# Autodesk Inventor assembly: Wobbler Assembly
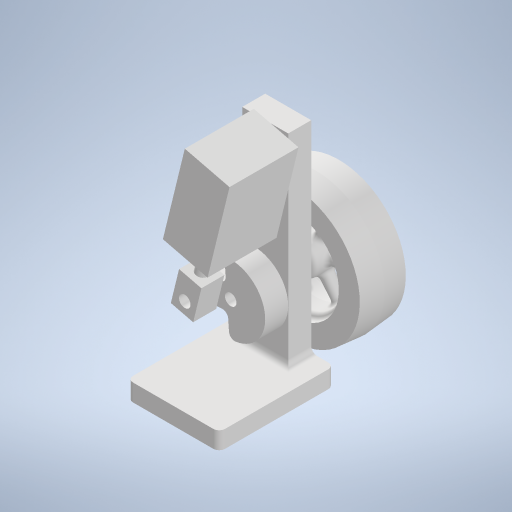
[picture p0: Inventor's stored thumbnail of the model, 512x512]
Saved by Autodesk Inventor 2023 (Build 270158000, 158)
## iProperties
Created: 2022-12-28
Part Number: Wobbler Assembly
Document SubType Name: Assembly
Designer: tgr41
Author: tgr41
## Documents named in this file (6)
- C:\Users\tommy\Documents\Repositories\Steam-Engine\Cast Wobbler\Wobbler Assembly.iam
- C:\Users\tommy\Documents\Repositories\Steam-Engine\Cast Wobbler\Crank.ipt
- C:\Users\tommy\Documents\Repositories\Steam-Engine\Cast Wobbler\Cylinder.ipt
- C:\Users\tommy\Documents\Repositories\Steam-Engine\Cast Wobbler\Flywheel.ipt
- C:\Users\tommy\Documents\Repositories\Steam-Engine\Cast Wobbler\Piston Assembly.ipt
- C:\Users\tommy\Documents\Repositories\Steam-Engine\Cast Wobbler\Based.ipt
## Components (5 placed, 5 different names)
1. Crank:1 — Mate:2, Mate:3, Mate:4, Angle:1
2. Cylinder:1 — Mate:5, Mate:6, Mate:7, Mate:8
3. Flywheel:1 — Mate:1, Mate:9, Angle:1
4. Based:1 — Mate:1, Mate:2, Mate:7, Mate:8, Mate:9
5. Piston Assembly:1 — Mate:3, Mate:4, Mate:5, Mate:6
## Relationships (10: Mate 9, Angle 1)
- Mate:1: Flywheel:1 ↔ Based:1
- Mate:2: Crank:1 ↔ Based:1
- Mate:3: Crank:1 ↔ Piston Assembly:1
- Mate:4: Crank:1 ↔ Piston Assembly:1
- Mate:5: Cylinder:1 ↔ Piston Assembly:1
- Mate:6: Cylinder:1 ↔ Piston Assembly:1
- Mate:7: Cylinder:1 ↔ Based:1
- Mate:8: Cylinder:1 ↔ Based:1
- Mate:9 (2.54 mm): Flywheel:1 ↔ Based:1
- Angle:1 (0 deg): Crank:1 ↔ Flywheel:1
